# Autodesk Inventor assembly: Drivetrain
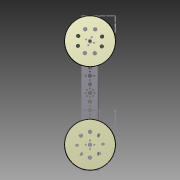
[picture p0: Inventor's stored thumbnail of the model, 180x180]
Saved by Autodesk Inventor 2014 SP2 (Build 180246200, 246)
## iProperties
Created: 2014-09-07
Part Number: Drivetrain
Document SubType Name: Assembly
Designer: Allison
Author: Allison
## Documents named in this file (6)
- C:\Users\Allison\Documents\inventor\InventorMasterProject\Drivetrain.iam
- C:\Users\Allison\Documents\Inventor\InventorMasterProject\Tetrix\Wheels\4 Inch Wheel.ipt
- C:\Users\Allison\Documents\Inventor\InventorMasterProject\Tetrix\Spacers\Hub Spacer.ipt
- C:\Users\Allison\Documents\Inventor\InventorMasterProject\Tetrix\Hubs and Axles\Bronze Bushing.ipt
- C:\Users\Allison\Documents\Inventor\InventorMasterProject\Drivetrain channel.ipt
- C:\Users\Allison\Documents\Inventor\InventorMasterProject\Special Drivetrain Channel.ipt
## Components (16 placed, 5 different names)
1. Special Drivetrain Channel:1 — Insert:30, Insert:31, Insert:32, Insert:44, Insert:45
2. 4 Inch Wheel:1 — Insert:9
3. Hub Spacer:1 — Insert:9, Insert:11
4. Bronze Bushing:1 — Insert:11, Insert:45
5. 4 Inch Wheel:2
6. Hub Spacer:2
7. Bronze Bushing:2 — Insert:44
8. Drivetrain channel:2 — Insert:31, Insert:32, Insert:33
9. Special Drivetrain Channel:2 — Insert:29, Insert:33, Insert:43, Insert:46, Insert:47
10. Drivetrain channel:3 — Insert:29, Insert:30, Insert:43
11. 4 Inch Wheel:3
12. Hub Spacer:3
13. Bronze Bushing:3 — Insert:46
14. 4 Inch Wheel:4
15. Hub Spacer:4
16. Bronze Bushing:4 — Insert:47
## Relationships (18: Insert 18)
- Insert:9: 4 Inch Wheel:1 ↔ Hub Spacer:1
- Insert:11: Hub Spacer:1 ↔ Bronze Bushing:1
- [Insert]: 4 Inch Wheel:2 ↔ Hub Spacer:2
- [Insert]: Hub Spacer:2 ↔ Bronze Bushing:2
- Insert:29: Special Drivetrain Channel:2 ↔ Drivetrain channel:3
- Insert:30: Special Drivetrain Channel:1 ↔ Drivetrain channel:3
- Insert:31: Special Drivetrain Channel:1 ↔ Drivetrain channel:2
- Insert:32: Special Drivetrain Channel:1 ↔ Drivetrain channel:2
- Insert:33: Drivetrain channel:2 ↔ Special Drivetrain Channel:2
- [Insert]: 4 Inch Wheel:3 ↔ Hub Spacer:3
- [Insert]: Hub Spacer:3 ↔ Bronze Bushing:3
- [Insert]: 4 Inch Wheel:4 ↔ Hub Spacer:4
- [Insert]: Hub Spacer:4 ↔ Bronze Bushing:4
- Insert:43: Special Drivetrain Channel:2 ↔ Drivetrain channel:3
- Insert:44: Special Drivetrain Channel:1 ↔ Bronze Bushing:2
- Insert:45: Special Drivetrain Channel:1 ↔ Bronze Bushing:1
- Insert:46: Special Drivetrain Channel:2 ↔ Bronze Bushing:3
- Insert:47: Special Drivetrain Channel:2 ↔ Bronze Bushing:4
## Named parameters: d32_d28 = 0 mm, d34_d30 = 0 mm, d76_d28 = 0 mm, d78_d30 = 0 mm, d80_d32_d28 = 0 mm, d82_d34_d30 = 0 mm
